# Autodesk Inventor assembly: model lathe
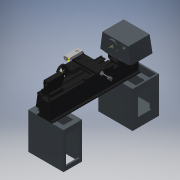
[picture p0: Inventor's stored thumbnail of the model, 180x180]
Saved by Autodesk Inventor 2016 (Build 200138000, 138)
## iProperties
Created: 2017-05-02
Part Number: model lathe
Document SubType Name: Assembly
Designer: M228544
Author: M228544
## Documents named in this file (13)
- C:\Users\M228544\x axis shaft.iam
- C:\Users\M228544\Term 2\BED.ipt
- C:\Users\M228544\Term 2\saddle.ipt
- C:\Users\M228544\Term 2\Bottom-Tool-Bit.ipt
- C:\Users\M228544\Term 2\Top-Part-Tool-bit.ipt
- C:\Users\M228544\Term 2\slide-ontop-of-saddle.ipt
- C:\Users\M228544\Term 2\tail stock - body part.ipt
- C:\Users\M228544\Term 2\Gearbox.ipt
- C:\Users\M228544\Term 2\Left leg.ipt
- C:\Users\M228544\Term 2\Right Leg.ipt
- C:\Users\M228544\Term 2\Apron.ipt
- C:\Users\M228544\Term 2\Ball screw support [bed].ipt
- C:\Users\M228544\shaft and nut.iam
## Components (12 placed, 12 different names)
1. BED:1 — Mate:1, Mate:2, Mate:9, Mate:10, Mate:11, Flush:5, Flush:6, Mate:13, Mate:14, Flush:7, Flush:9, Mate:16, Mate:17, Mate:18
2. saddle:1 — Mate:1, Mate:2, Mate:5, Mate:6, Saddle and Slice on top of saddle, Flush:10, Flush:11, Mate:15, Mate:20, Mate:22, Mate:24
3. Bottom-Tool-Bit:1 — Mate:3, Mate:4, Flush:14
4. Top-Part-Tool-bit:1 — Mate:3, Mate:4, Mate:7, Mate:8, Tool Bit and Slece on top of saddle, Flush:14
5. slide-ontop-of-saddle:1 — Mate:5, Mate:6, Mate:7, Mate:8, Saddle and Slice on top of saddle, Tool Bit and Slece on top of saddle, Mate:23
6. tail stock - body part:1 — Mate:9, Mate:10, Flush:13, Mate:19, Mate:20
7. Gearbox:1 — Mate:11, Flush:5, Flush:13, Mate:19, Mate:21
8. Left leg:1 — Mate:14, Flush:7, Flush:8
9. Right Leg:1 — Flush:6, Mate:13, Flush:8, Flush:9
10. Apron:1 — Flush:10, Flush:11, Mate:15, Mate:21
11. Ball screw support [bed]:1 — Mate:16, Mate:17, Mate:18
12. shaft and nut:1 [sub-assembly] — Mate:22, Mate:23, Mate:24
## Relationships (34: Mate 23, Flush 10, Angle 1)
- Mate:1: BED:1 ↔ saddle:1
- Mate:2: BED:1 ↔ saddle:1
- Mate:3: Bottom-Tool-Bit:1 ↔ Top-Part-Tool-bit:1
- Mate:4: Bottom-Tool-Bit:1 ↔ Top-Part-Tool-bit:1
- Mate:5: saddle:1 ↔ slide-ontop-of-saddle:1
- Mate:6: saddle:1 ↔ slide-ontop-of-saddle:1
- Mate:7: Top-Part-Tool-bit:1 ↔ slide-ontop-of-saddle:1
- Mate:8: Top-Part-Tool-bit:1 ↔ slide-ontop-of-saddle:1
- Mate:9: BED:1 ↔ tail stock - body part:1
- Mate:10: BED:1 ↔ tail stock - body part:1
- Saddle and Slice on top of saddle [Flush]: saddle:1 ↔ slide-ontop-of-saddle:1
- Tool Bit and Slece on top of saddle [Angle] (-90 deg): Top-Part-Tool-bit:1 ↔ slide-ontop-of-saddle:1
- Mate:11: BED:1 ↔ Gearbox:1
- Flush:5: BED:1 ↔ Gearbox:1
- Flush:13: tail stock - body part:1 ↔ Gearbox:1
- Flush:6: BED:1 ↔ Right Leg:1
- Mate:13: BED:1 ↔ Right Leg:1
- Mate:14: BED:1 ↔ Left leg:1
- Flush:7: BED:1 ↔ Left leg:1
- Flush:8: Left leg:1 ↔ Right Leg:1
- Flush:9 (145 mm): BED:1 ↔ Right Leg:1
- Flush:10: saddle:1 ↔ Apron:1
- Flush:11: saddle:1 ↔ Apron:1
- Mate:15: saddle:1 ↔ Apron:1
- Mate:16: BED:1 ↔ Ball screw support [bed]:1
- Mate:17: BED:1 ↔ Ball screw support [bed]:1
- Mate:18: BED:1 ↔ Ball screw support [bed]:1
- Flush:14: Bottom-Tool-Bit:1 ↔ Top-Part-Tool-bit:1
- Mate:19: tail stock - body part:1 ↔ Gearbox:1
- Mate:20: saddle:1 ↔ tail stock - body part:1
- Mate:21: Gearbox:1 ↔ Apron:1
- Mate:22: saddle:1 ↔ shaft and nut:1
- Mate:23: slide-ontop-of-saddle:1 ↔ shaft and nut:1
- Mate:24: saddle:1 ↔ shaft and nut:1
